# Autodesk Inventor assembly: Claw
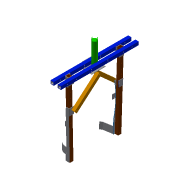
[picture p0: Inventor's stored thumbnail of the model, 180x180]
Saved by Autodesk Inventor 2015 (Build 190159000, 159)
## iProperties
Created: 2015-01-13
Part Number: Claw
Document SubType Name: Assembly
Designer: Collin_2
Author: Collin_2
## Documents named in this file (17)
- C:\Users\Tanner\Documents\GitHub\FIRST-Team-1719-CAD-Team\2015 Robot CAD\Devices\Claw\Claw.iam
- C:\Users\Tanner\Documents\GitHub\FIRST-Team-1719-CAD-Team\2015 Robot CAD\Devices\Claw\Claw - Base.ipt
- C:\Users\Tanner\Documents\GitHub\FIRST-Team-1719-CAD-Team\2015 Robot CAD\Devices\Claw\PC3.5-P1.ipt
- C:\Users\Tanner\Documents\GitHub\FIRST-Team-1719-CAD-Team\2015 Robot CAD\Devices\Claw\PC3.5-ROD.ipt
- C:\Users\Tanner\Documents\GitHub\FIRST-Team-1719-CAD-Team\2015 Robot CAD\Devices\Claw\Claw - Arm - Middle.ipt
- C:\Users\Tanner\Documents\GitHub\FIRST-Team-1719-CAD-Team\2015 Robot CAD\Devices\Claw\Yarm.ipt
- C:\Users\Tanner\Documents\GitHub\FIRST-Team-1719-CAD-Team\2015 Robot CAD\Devices\Claw\Claw - L bracket.ipt
- C:\Users\Tanner\Documents\GitHub\FIRST-Team-1719-CAD-Team\2015 Robot CAD\Devices\Claw\Claw - Arm - Plate 2.ipt
- C:\Users\Tanner\Documents\GitHub\FIRST-Team-1719-CAD-Team\2015 Robot CAD\Devices\Claw\Claw - End piece.ipt
- C:\Users\Tanner\Documents\GitHub\FIRST-Team-1719-CAD-Team\2015 Robot CAD\Devices\Claw\Claw - Arm - Top (R) v2.ipt
- C:\Users\Tanner\Documents\GitHub\FIRST-Team-1719-CAD-Team\2015 Robot CAD\Devices\Claw\Claw - Arm - Bottom (R) v2.ipt
- C:\Users\Tanner\Documents\GitHub\FIRST-Team-1719-CAD-Team\2015 Robot CAD\Devices\Claw\Claw - Arm - Bottom (R) v3.ipt
- C:\Users\Tanner\Documents\GitHub\FIRST-Team-1719-CAD-Team\2015 Robot CAD\Devices\Claw\Claw - Arm - Top (R) v3.ipt
- C:\Users\Tanner\Documents\GitHub\FIRST-Team-1719-CAD-Team\2015 Robot CAD\Devices\Claw\Claw - Arm - Bottom  (R) - Top.ipt
- C:\Users\Tanner\Documents\GitHub\FIRST-Team-1719-CAD-Team\2015 Robot CAD\Devices\Claw\Claw - Arm - Bottom (R) Bottom.ipt
- C:\Users\Tanner\Documents\GitHub\FIRST-Team-1719-CAD-Team\2015 Robot CAD\Devices\Claw\Claw - Arm - Top (R) Bottom.ipt
- C:\Users\Tanner\Documents\GitHub\FIRST-Team-1719-CAD-Team\2015 Robot CAD\Devices\Claw\Claw - Arm - Top (R) Top.ipt
## Components (21 placed, 16 different names)
1. Claw - Base:1 — Tangent:2, Flush:8, Mate:52, Flush:9, Flush:10, Flush:11, Flush:26, Mate:94
2. PC3.5-P1:1 — Mate:15, Mate:16, Tangent:2, Mate:53
3. PC3.5-ROD:1 — Mate:15, Mate:16, Mate:37, Mate:55
4. Claw - Arm - Middle:1 — Mate:58, Mate:59, Mate:65, Flush:12, Mate:69, Mate:70, Flush:23, Mate:84, Mate:89, Flush:25, Mate:90
5. Claw - Arm - Middle:2 — Mate:63, Flush:14, Mate:73, Mate:74, Mate:75, Flush:22, Mate:82, Mate:83, Mate:86, Mate:87
6. Yarm:1 — Mate:37, Mate:40, Insert:3
7. Yarm:2 — Mate:40, Mate:55, Insert:4
8. Claw - L bracket:1 — Flush:8, Mate:52, Mate:53, Flush:11
9. Claw - Base:2 — Flush:9, Flush:10, Mate:67, Mate:68, Mate:91, Mate:92, Flush:26, Mate:93
10. Claw - Arm - Plate 2:1 — Insert:6, Angle:2
11. Claw - Arm - Plate 2:2 — Insert:5, Angle:1
12. Claw - End piece:1 — Flush:20, Flush:21, Mate:80
13. Claw - End piece:2 — Mate:79, Flush:18, Flush:19
14. Claw - Arm - Top (R) v2:1 — Mate:58, Mate:59, Insert:3, Mate:96
15. Claw - Arm - Bottom (R) v2:1 — Mate:82, Mate:83, Mate:95
16. Claw - Arm - Bottom (R) v3:1 — Mate:63, Mate:67, Mate:75, Flush:22, Flush:24, Mate:92, Mate:93
17. Claw - Arm - Top (R) v3:1 — Mate:65, Mate:68, Flush:23, Mate:84
18. Claw - Arm - Bottom (R) Bottom:1 — Flush:12, Mate:69, Mate:70, Flush:20, Flush:21, Mate:80, Mate:96, Insert:6, Angle:2
19. Claw - Arm - Top (R) Bottom:1 — Flush:14, Mate:73, Mate:74, Mate:79, Flush:18, Flush:19, Insert:4, Mate:95, Insert:5, Angle:1
20. Claw - Arm - Bottom  (R) - Top:1 — Flush:24, Mate:86, Mate:87, Mate:94
21. Claw - Arm - Top (R) Top:2 — Mate:89, Flush:25, Mate:90, Mate:91
## Relationships (55: Mate 33, Flush 15, Insert 4, Angle 2, Tangent 1)
- Mate:15: PC3.5-P1:1 ↔ PC3.5-ROD:1
- Mate:16: PC3.5-P1:1 ↔ PC3.5-ROD:1
- Mate:37: PC3.5-ROD:1 ↔ Yarm:1
- Mate:40: Yarm:1 ↔ Yarm:2
- Tangent:2 (285.75 mm): Claw - Base:1 ↔ PC3.5-P1:1
- Flush:8: Claw - Base:1 ↔ Claw - L bracket:1
- Mate:52: Claw - Base:1 ↔ Claw - L bracket:1
- Mate:53: PC3.5-P1:1 ↔ Claw - L bracket:1
- Flush:9: Claw - Base:1 ↔ Claw - Base:2
- Flush:10: Claw - Base:1 ↔ Claw - Base:2
- Mate:55: PC3.5-ROD:1 ↔ Yarm:2
- Flush:11 (-250.825 mm): Claw - Base:1 ↔ Claw - L bracket:1
- Mate:58: Claw - Arm - Middle:1 ↔ Claw - Arm - Top (R) v2:1
- Mate:59: Claw - Arm - Middle:1 ↔ Claw - Arm - Top (R) v2:1
- Mate:63: Claw - Arm - Middle:2 ↔ Claw - Arm - Bottom (R) v3:1
- Mate:65: Claw - Arm - Middle:1 ↔ Claw - Arm - Top (R) v3:1
- Mate:67: Claw - Base:2 ↔ Claw - Arm - Bottom (R) v3:1
- Mate:68: Claw - Base:2 ↔ Claw - Arm - Top (R) v3:1
- Flush:12: Claw - Arm - Middle:1 ↔ Claw - Arm - Bottom (R) Bottom:1
- Mate:69: Claw - Arm - Middle:1 ↔ Claw - Arm - Bottom (R) Bottom:1
- Mate:70: Claw - Arm - Middle:1 ↔ Claw - Arm - Bottom (R) Bottom:1
- Flush:14: Claw - Arm - Middle:2 ↔ Claw - Arm - Top (R) Bottom:1
- Mate:73: Claw - Arm - Middle:2 ↔ Claw - Arm - Top (R) Bottom:1
- Mate:74: Claw - Arm - Middle:2 ↔ Claw - Arm - Top (R) Bottom:1
- Mate:75: Claw - Arm - Middle:2 ↔ Claw - Arm - Bottom (R) v3:1
- Mate:79: Claw - End piece:2 ↔ Claw - Arm - Top (R) Bottom:1
- Flush:18: Claw - End piece:2 ↔ Claw - Arm - Top (R) Bottom:1
- Flush:19: Claw - End piece:2 ↔ Claw - Arm - Top (R) Bottom:1
- Flush:20: Claw - End piece:1 ↔ Claw - Arm - Bottom (R) Bottom:1
- Flush:21: Claw - End piece:1 ↔ Claw - Arm - Bottom (R) Bottom:1
- Mate:80: Claw - End piece:1 ↔ Claw - Arm - Bottom (R) Bottom:1
- Flush:22: Claw - Arm - Middle:2 ↔ Claw - Arm - Bottom (R) v3:1
- Mate:82: Claw - Arm - Middle:2 ↔ Claw - Arm - Bottom (R) v2:1
- Mate:83: Claw - Arm - Middle:2 ↔ Claw - Arm - Bottom (R) v2:1
- Flush:23: Claw - Arm - Middle:1 ↔ Claw - Arm - Top (R) v3:1
- Mate:84: Claw - Arm - Middle:1 ↔ Claw - Arm - Top (R) v3:1
- Flush:24: Claw - Arm - Bottom (R) v3:1 ↔ Claw - Arm - Bottom  (R) - Top:1
- Mate:86: Claw - Arm - Middle:2 ↔ Claw - Arm - Bottom  (R) - Top:1
- Mate:87: Claw - Arm - Middle:2 ↔ Claw - Arm - Bottom  (R) - Top:1
- Mate:89: Claw - Arm - Middle:1 ↔ Claw - Arm - Top (R) Top:2
- Flush:25: Claw - Arm - Middle:1 ↔ Claw - Arm - Top (R) Top:2
- Mate:90: Claw - Arm - Middle:1 ↔ Claw - Arm - Top (R) Top:2
- Mate:91: Claw - Base:2 ↔ Claw - Arm - Top (R) Top:2
- Mate:92: Claw - Base:2 ↔ Claw - Arm - Bottom (R) v3:1
- Insert:3: Yarm:1 ↔ Claw - Arm - Top (R) v2:1
- Insert:4: Yarm:2 ↔ Claw - Arm - Top (R) Bottom:1
- Flush:26: Claw - Base:1 ↔ Claw - Base:2
- Mate:93: Claw - Base:2 ↔ Claw - Arm - Bottom (R) v3:1
- Mate:94: Claw - Base:1 ↔ Claw - Arm - Bottom  (R) - Top:1
- Mate:95: Claw - Arm - Bottom (R) v2:1 ↔ Claw - Arm - Top (R) Bottom:1
- Mate:96: Claw - Arm - Top (R) v2:1 ↔ Claw - Arm - Bottom (R) Bottom:1
- Insert:5: Claw - Arm - Plate 2:2 ↔ Claw - Arm - Top (R) Bottom:1
- Angle:1 (0 deg): Claw - Arm - Plate 2:2 ↔ Claw - Arm - Top (R) Bottom:1
- Insert:6: Claw - Arm - Plate 2:1 ↔ Claw - Arm - Bottom (R) Bottom:1
- Angle:2 (0 deg): Claw - Arm - Plate 2:1 ↔ Claw - Arm - Bottom (R) Bottom:1
